# Autodesk Inventor assembly: Re-entrant Flange
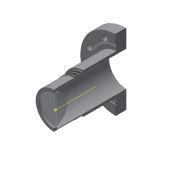
[picture p0: Inventor's stored thumbnail of the model, 180x180]
Saved by Autodesk Inventor 2015 SP1 (Build 190203100, 203)
## iProperties
Created: 2014-07-08
Part Number: Re-entrant Flange
Document SubType Name: Assembly
Designer: I Rabey
Author: I Rabey
## Documents named in this file (6)
- C:\ColdMatter\CADFiles\EDM Machine\Detection Region\Re-entrant Flange and Mirrors\Re-entrant Flange.iam
- C:\ColdMatter\CADFiles\EDM Machine\Detection Region\Re-entrant Flange and Mirrors\Vacuum Cylinder.ipt
- C:\ColdMatter\CADFiles\EDM Machine\Detection Region\Re-entrant Flange and Mirrors\DN63CF Counter Bored.ipt
- C:\ColdMatter\CADFiles\EDM Machine\Detection Region\Re-entrant Flange and Mirrors\Cap.ipt
- C:\ColdMatter\CADFiles\EDM Machine\Detection Region\Re-entrant Flange and Mirrors\Comar39AF50.ipt
- C:\ColdMatter\CADFiles\EDM Machine\Detection Region\Re-entrant Flange and Mirrors\Window Comar 50GJ03.ipt
## Components (5 placed, 5 different names)
1. DN63CF Counter Bored:1 — Mate:1, Mate:2, Mate:3, Mate:4
2. Vacuum Cylinder:1 — Mate:3, Mate:4, Mate:11, Mate:12, Mate:15, Mate:20, Mate:21
3. Cap:1 — Mate:11, Mate:12, Mate:13, Mate:16, Mate:17, Mate:20, Mate:22
4. Window Comar 50GJ03:1 — Mate:15, Mate:16, Mate:17
5. Comar39AF50:1 — Mate:21, Mate:22
## Relationships (13: Mate 13)
- Mate:1: DN63CF Counter Bored:1
- Mate:2: DN63CF Counter Bored:1
- Mate:3: DN63CF Counter Bored:1 ↔ Vacuum Cylinder:1
- Mate:4: DN63CF Counter Bored:1 ↔ Vacuum Cylinder:1
- Mate:11: Vacuum Cylinder:1 ↔ Cap:1
- Mate:12: Vacuum Cylinder:1 ↔ Cap:1
- Mate:13: Cap:1
- Mate:15: Vacuum Cylinder:1 ↔ Window Comar 50GJ03:1
- Mate:16: Cap:1 ↔ Window Comar 50GJ03:1
- Mate:17: Cap:1 ↔ Window Comar 50GJ03:1
- Mate:20: Vacuum Cylinder:1 ↔ Cap:1
- Mate:21: Vacuum Cylinder:1 ↔ Comar39AF50:1
- Mate:22: Cap:1 ↔ Comar39AF50:1
